# Autodesk Inventor assembly: каретка
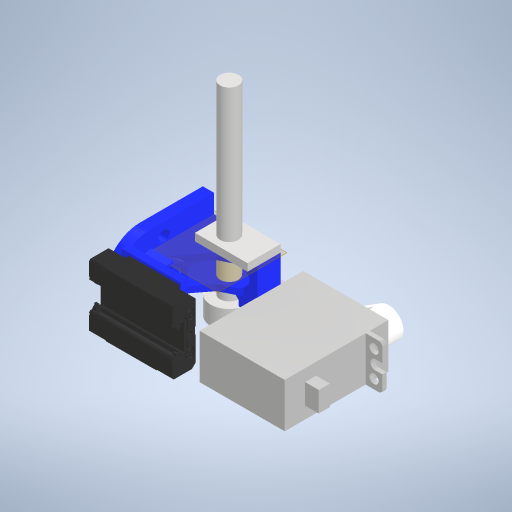
[picture p0: Inventor's stored thumbnail of the model, 512x512]
Saved by Autodesk Inventor 2024.2 (Build 282272000, 272)
## iProperties
Created: 2026-01-30
Part Number: каретка
Document SubType Name: Assembly
Designer: Service
Author: Service
## Documents named in this file (8)
- C:\Users\Service\Documents\Artist-v2\3D\каретка.iam
- C:\Users\Service\Documents\Artist-v2\3D\крепежная основа.ipt
- C:\Users\Service\Documents\Artist-v2\3D\MGN7C_MGN7C.ipt
- C:\Users\Service\Documents\Artist\3D\стл\Сборка плоттер\Сервопривод.ipt
- C:\Users\Service\Documents\Artist\3D\стл\Сборка плоттер\Деталь.ipt
- C:\Users\Service\Documents\Artist-v2\3D\stl\вал с пружиной.ipt
- C:\Users\Service\Documents\Artist-v2\3D\stl\каретка.ipt
- C:\Users\Service\Documents\Artist-v2\3D\MGN7.ipt
## Components (7 placed, 7 different names)
1. крепежная основа:1 — Совмещение:1, Заподлицо:1, Совмещение:7, Совмещение:8, Совмещение:11
2. MGN7C_MGN7C:1 — Совмещение:1
3. Сервопривод:1 — Совмещение:4, Совмещение:5, Совмещение:11
4. Деталь:1 — Совмещение:4, Совмещение:5
5. вал с пружиной:1 — Совмещение:7
6. каретка:1 — Заподлицо:1
7. MGN7:1 — Совмещение:8
## Relationships (7: Mate 6, Flush 1)
- Совмещение:1 [Mate]: крепежная основа:1 ↔ MGN7C_MGN7C:1
- Совмещение:4 [Mate]: Сервопривод:1 ↔ Деталь:1
- Совмещение:5 [Mate]: Сервопривод:1 ↔ Деталь:1
- Заподлицо:1 [Flush]: крепежная основа:1 ↔ каретка:1
- Совмещение:7 [Mate]: крепежная основа:1 ↔ вал с пружиной:1
- Совмещение:8 [Mate]: крепежная основа:1 ↔ MGN7:1
- Совмещение:11 [Mate]: крепежная основа:1 ↔ Сервопривод:1
